# Autodesk Inventor assembly: NanoPower P31u-9
(part 2 of 2)
- C:\Users\Cosmonauta\ownCloud\Aurora\Proyectos\SUCHAI_2-3\Subsistemas\MEC\CAD_Cubesat3U\Nanopower_P31U\CAD\U7.iam
- C:\Users\Cosmonauta\ownCloud\Aurora\Proyectos\SUCHAI_2-3\Subsistemas\MEC\CAD_Cubesat3U\Nanopower_P31U\CAD\Y2.iam
- C:\Users\Cosmonauta\ownCloud\Aurora\Proyectos\SUCHAI_2-3\Subsistemas\MEC\CAD_Cubesat3U\Nanopower_P31U\CAD\Q1.iam
- C:\Users\Cosmonauta\ownCloud\Aurora\Proyectos\SUCHAI_2-3\Subsistemas\MEC\CAD_Cubesat3U\Nanopower_P31U\CAD\R22.iam
- C:\Users\Cosmonauta\ownCloud\Aurora\Proyectos\SUCHAI_2-3\Subsistemas\MEC\CAD_Cubesat3U\Nanopower_P31U\CAD\R23.iam
- C:\Users\Cosmonauta\ownCloud\Aurora\Proyectos\SUCHAI_2-3\Subsistemas\MEC\CAD_Cubesat3U\Nanopower_P31U\CAD\Free-Models.iam
## Components (321 placed, 321 different names)
1. 66
2. 69 [sub-assembly]
3. 75 [sub-assembly]
4. 78 [sub-assembly]
5. 82 [sub-assembly]
6. 85 [sub-assembly]
7. 88 [sub-assembly]
8. 90 [sub-assembly]
9. 93 [sub-assembly]
10. 96 [sub-assembly]
11. 98 [sub-assembly]
12. 100 [sub-assembly]
13. 102 [sub-assembly]
14. 104 [sub-assembly]
15. 106 [sub-assembly]
16. 109 [sub-assembly]
17. 111 [sub-assembly]
18. 113 [sub-assembly]
19. 115 [sub-assembly]
20. 117 [sub-assembly]
21. 123 [sub-assembly]
22. 129 [sub-assembly]
23. 133 [sub-assembly]
24. 137 [sub-assembly]
25. 141 [sub-assembly]
26. 145 [sub-assembly]
27. 147 [sub-assembly]
28. 149 [sub-assembly]
29. 151 [sub-assembly]
30. 154 [sub-assembly]
31. 156 [sub-assembly]
32. 158 [sub-assembly]
33. 160 [sub-assembly]
34. 162 [sub-assembly]
35. 164 [sub-assembly]
36. 166 [sub-assembly]
37. 168 [sub-assembly]
38. 170 [sub-assembly]
39. 172 [sub-assembly]
40. 174 [sub-assembly]
41. 176 [sub-assembly]
42. 178 [sub-assembly]
43. 181 [sub-assembly]
44. 185 [sub-assembly]
45. 188 [sub-assembly]
46. 190 [sub-assembly]
47. 193 [sub-assembly]
48. 196 [sub-assembly]
49. 198 [sub-assembly]
50. 200 [sub-assembly]
51. 202 [sub-assembly]
52. 204 [sub-assembly]
53. 206 [sub-assembly]
54. 214 [sub-assembly]
55. 216 [sub-assembly]
56. 218 [sub-assembly]
57. 225 [sub-assembly]
58. 229 [sub-assembly]
59. 233 [sub-assembly]
60. 235 [sub-assembly]
61. 237 [sub-assembly]
62. 239 [sub-assembly]
63. 241 [sub-assembly]
64. 243 [sub-assembly]
65. 245 [sub-assembly]
66. 247 [sub-assembly]
67. 249 [sub-assembly]
68. 251 [sub-assembly]
69. 253 [sub-assembly]
70. 257 [sub-assembly]
71. 261 [sub-assembly]
72. 268 [sub-assembly]
73. 272 [sub-assembly]
74. 274 [sub-assembly]
75. 276 [sub-assembly]
76. 278 [sub-assembly]
77. 280 [sub-assembly]
78. 283 [sub-assembly]
79. 285 [sub-assembly]
80. 287 [sub-assembly]
81. 289 [sub-assembly]
82. 291 [sub-assembly]
83. 294 [sub-assembly]
84. 296 [sub-assembly]
85. 298 [sub-assembly]
86. 300 [sub-assembly]
87. 302 [sub-assembly]
88. 304 [sub-assembly]
89. 306 [sub-assembly]
90. 308 [sub-assembly]
91. 310 [sub-assembly]
92. 312 [sub-assembly]
93. 314 [sub-assembly]
94. 316 [sub-assembly]
95. 319 [sub-assembly]
96. 321 [sub-assembly]
97. 323 [sub-assembly]
98. 326 [sub-assembly]
99. 328 [sub-assembly]
100. 330 [sub-assembly]
101. 332 [sub-assembly]
102. 335 [sub-assembly]
103. 337 [sub-assembly]
104. 339 [sub-assembly]
105. 341 [sub-assembly]
106. 343 [sub-assembly]
107. 345 [sub-assembly]
108. 347 [sub-assembly]
109. 349 [sub-assembly]
110. 351 [sub-assembly]
111. 353 [sub-assembly]
112. 355 [sub-assembly]
113. 357 [sub-assembly]
114. 359 [sub-assembly]
115. 361 [sub-assembly]
116. 363 [sub-assembly]
117. 365 [sub-assembly]
118. 367 [sub-assembly]
119. 369 [sub-assembly]
120. 371 [sub-assembly]
121. 373 [sub-assembly]
122. 375 [sub-assembly]
123. 377 [sub-assembly]
124. 379 [sub-assembly]
125. 381 [sub-assembly]
126. 383 [sub-assembly]
127. 385 [sub-assembly]
128. 388 [sub-assembly]
129. 391 [sub-assembly]
130. 394 [sub-assembly]
131. 396 [sub-assembly]
132. 398 [sub-assembly]
133. 400 [sub-assembly]
134. 402 [sub-assembly]
135. 404 [sub-assembly]
136. 406 [sub-assembly]
137. 408 [sub-assembly]
138. 410 [sub-assembly]
139. 412 [sub-assembly]
140. 414 [sub-assembly]
141. 416 [sub-assembly]
142. 418 [sub-assembly]
143. 420 [sub-assembly]
144. 422 [sub-assembly]
145. 424 [sub-assembly]
146. 426 [sub-assembly]
147. 428 [sub-assembly]
148. 430 [sub-assembly]
149. 432 [sub-assembly]
150. 434 [sub-assembly]
151. 436 [sub-assembly]
152. 438 [sub-assembly]
153. 440 [sub-assembly]
154. 442 [sub-assembly]
155. 444 [sub-assembly]
156. 447 [sub-assembly]
157. 449 [sub-assembly]
158. 451 [sub-assembly]
159. 461 [sub-assembly]
160. 463 [sub-assembly]
161. 465 [sub-assembly]
162. 467 [sub-assembly]
163. 469 [sub-assembly]
164. 471 [sub-assembly]
165. 473 [sub-assembly]
166. 476 [sub-assembly]
167. 478 [sub-assembly]
168. 481 [sub-assembly]
169. 483 [sub-assembly]
170. 485 [sub-assembly]
171. 487 [sub-assembly]
172. 489 [sub-assembly]
173. 491 [sub-assembly]
174. 495 [sub-assembly]
175. 499 [sub-assembly]
176. 503 [sub-assembly]
177. 507 [sub-assembly]
178. 511 [sub-assembly]
179. 515 [sub-assembly]
180. 519 [sub-assembly]
181. 523 [sub-assembly]
182. 527 [sub-assembly]
183. 531 [sub-assembly]
184. 535 [sub-assembly]
185. 539 [sub-assembly]
186. 543 [sub-assembly]
187. 547 [sub-assembly]
188. 551 [sub-assembly]
189. 555 [sub-assembly]
190. 559 [sub-assembly]
191. 563 [sub-assembly]
192. 567 [sub-assembly]
193. 571 [sub-assembly]
194. 575 [sub-assembly]
195. 579 [sub-assembly]
196. 583 [sub-assembly]
197. 587 [sub-assembly]
198. 589 [sub-assembly]
199. 591 [sub-assembly]
200. 593 [sub-assembly]
201. 595 [sub-assembly]
202. 597 [sub-assembly]
203. 599 [sub-assembly]
204. 601 [sub-assembly]
205. 603 [sub-assembly]
206. 605 [sub-assembly]
207. 607 [sub-assembly]
208. 609 [sub-assembly]
209. 611 [sub-assembly]
210. 613 [sub-assembly]
211. 615 [sub-assembly]
212. 617 [sub-assembly]
213. 619 [sub-assembly]
214. 621 [sub-assembly]
215. 623 [sub-assembly]
216. 625 [sub-assembly]
217. 627 [sub-assembly]
218. 629 [sub-assembly]
219. 631 [sub-assembly]
220. 633 [sub-assembly]
221. 635 [sub-assembly]
222. 637 [sub-assembly]
223. 639 [sub-assembly]
224. 641 [sub-assembly]
225. 643 [sub-assembly]
226. 645 [sub-assembly]
227. 647 [sub-assembly]
228. 649 [sub-assembly]
229. 651 [sub-assembly]
230. 654 [sub-assembly]
231. 656 [sub-assembly]
232. 658 [sub-assembly]
233. 660 [sub-assembly]
234. 662 [sub-assembly]
235. 664 [sub-assembly]
236. 666 [sub-assembly]
237. 668 [sub-assembly]
238. 670 [sub-assembly]
239. 672 [sub-assembly]
240. 674 [sub-assembly]
241. 676 [sub-assembly]
242. 678 [sub-assembly]
243. 680 [sub-assembly]
244. 682 [sub-assembly]
245. 684 [sub-assembly]
246. 686 [sub-assembly]
247. 688 [sub-assembly]
248. 691 [sub-assembly]
249. 694 [sub-assembly]
250. 697 [sub-assembly]
251. 699 [sub-assembly]
252. 701 [sub-assembly]
253. 703 [sub-assembly]
254. 705 [sub-assembly]
255. 707 [sub-assembly]
256. 709 [sub-assembly]
257. 711 [sub-assembly]
258. 713 [sub-assembly]
259. 715 [sub-assembly]
260. 717 [sub-assembly]
261. 720 [sub-assembly]
262. 723 [sub-assembly]
263. 725 [sub-assembly]
264. 727 [sub-assembly]
265. 730 [sub-assembly]
266. 732 [sub-assembly]
267. 734 [sub-assembly]
268. 736 [sub-assembly]
269. 738 [sub-assembly]
270. 740 [sub-assembly]
271. 742 [sub-assembly]
272. 746 [sub-assembly]
273. 748 [sub-assembly]
274. 750 [sub-assembly]
275. 752 [sub-assembly]
276. 754 [sub-assembly]
277. 756 [sub-assembly]
278. 758 [sub-assembly]
279. 760 [sub-assembly]
280. 762 [sub-assembly]
281. 766 [sub-assembly]
282. 768 [sub-assembly]
283. 770 [sub-assembly]
284. 772 [sub-assembly]
285. 774 [sub-assembly]
286. 776 [sub-assembly]
287. 778 [sub-assembly]
288. 780 [sub-assembly]
289. 782 [sub-assembly]
290. 784 [sub-assembly]
291. 786 [sub-assembly]
292. 788 [sub-assembly]
293. 790 [sub-assembly]
294. 792 [sub-assembly]
295. 795 [sub-assembly]
296. 797 [sub-assembly]
297. 799 [sub-assembly]
298. 824 [sub-assembly]
299. 826 [sub-assembly]
300. 828 [sub-assembly]
301. 830 [sub-assembly]
302. 832 [sub-assembly]
303. 843 [sub-assembly]
304. 845 [sub-assembly]
305. 847 [sub-assembly]
306. 849 [sub-assembly]
307. 852 [sub-assembly]
308. 854 [sub-assembly]
309. 856 [sub-assembly]
310. 859 [sub-assembly]
311. 865 [sub-assembly]
312. 868 [sub-assembly]
313. 871 [sub-assembly]
314. 874 [sub-assembly]
315. 876 [sub-assembly]
316. 878 [sub-assembly]
317. 881 [sub-assembly]
318. 883 [sub-assembly]
319. 886 [sub-assembly]
320. 889 [sub-assembly]
321. 891 [sub-assembly]
